# Autodesk Inventor assembly: CARRITO
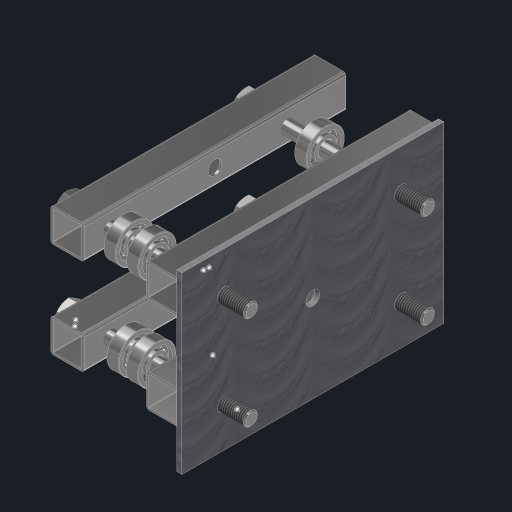
[picture p0: Inventor's stored thumbnail of the model, 512x512]
Saved by Autodesk Inventor 2024.3 (Build 283343000, 343)
## iProperties
Created: 2024-06-03
Part Number: CARRITO
Material: Generic
Document SubType Name: Assembly
Designer: Niler
_SolveAssemblyDoc: Frame Generator Solve Assembly
_Version: 25.0.0
Author: Niler
## Documents named in this file (12)
- C:\Users\Niler\OneDrive\Escritorio\RECICLADOR\RECICLADOR_MODELO_3D\CORTADORA_RECTA_2M\CARRITO.iam
- C:\Users\Niler\OneDrive\Escritorio\RECICLADOR\RECICLADOR_MODELO_3D\CORTADORA_RECTA_2M\CORTADORA_RECTA\Frame\AISC (1 1_4x1 1_4x1_8) 1717303404279.ipt
- C:\Users\Niler\OneDrive\Escritorio\RECICLADOR\RECICLADOR_MODELO_3D\CORTADORA_RECTA_2M\ESQUELETO_CARRITO.ipt
- C:\Users\Niler\OneDrive\Escritorio\RECICLADOR\RECICLADOR_MODELO_3D\CORTADORA_RECTA_2M\CARRITO\Frame\Frame 1717436838067.iam
- C:\Users\Niler\OneDrive\Escritorio\RECICLADOR\RECICLADOR_MODELO_3D\CORTADORA_RECTA_2M\CARRITO\Design Accelerator\Bearing1.iam
- C:\Users\Niler\OneDrive\Escritorio\RECICLADOR\RECICLADOR_MODELO_3D\LIBRERIA\en-US\AS 1111\AS 1111 - M8 x 100.ipt
- C:\Users\Niler\OneDrive\Escritorio\RECICLADOR\RECICLADOR_MODELO_3D\CORTADORA_RECTA_2M\CARRITO\Design Accelerator\Bearing2.iam
- C:\Users\Niler\OneDrive\Escritorio\RECICLADOR\RECICLADOR_MODELO_3D\CORTADORA_RECTA_2M\CARRITO\Design Accelerator\Bearing5.iam
- C:\Users\Niler\OneDrive\Escritorio\RECICLADOR\RECICLADOR_MODELO_3D\CORTADORA_RECTA_2M\CARRITO\Design Accelerator\Bearing6.iam
- C:\Users\Niler\OneDrive\Escritorio\RECICLADOR\RECICLADOR_MODELO_3D\LIBRERIA\en-US\AS 1111\AS 1111 - M8 x 50.ipt
- C:\Users\Niler\OneDrive\Escritorio\RECICLADOR\RECICLADOR_MODELO_3D\CORTADORA_RECTA_2M\PLACA.ipt
- C:\Users\Niler\OneDrive\Escritorio\RECICLADOR\RECICLADOR_MODELO_3D\LIBRERIA\en-US\ANSI B18.2.4.2M\ANSI B18.2.4.2M - M8x1.25 - 13.ipt
## Components (23 placed, 8 different names)
1. AISC (1 1/4x1 1/4x1/8) - 66.929:1 — Mate:1, Mate:2, Flush:1, Tangent:1, Tangent:2, Tangent:3, Tangent:4, Tangent:5
2. ESQUELETO_CARRITO:1
3. Frame 1717436838067:1 [sub-assembly] — Mate:6, Mate:7, Mate:13, Mate:15, Mate:17, Mate:23, Mate:24, Mate:28, Mate:31, Mate:33, Mate:35, Mate:37
4. Bearing:1 [sub-assembly] — Tangent:1, Mate:3
5. Bearing:2 [sub-assembly] — Tangent:2, Mate:4
6. AS 1111 - Metric M8 x 100:1 — Mate:3, Mate:4, Mate:6, Mate:13, Mate:25, Mate:30
7. Bearing:3 [sub-assembly]
8. Bearing:4 [sub-assembly]
9. AS 1111 - Metric M8 x 100:2 — Mate:7, Mate:8, Mate:26, Mate:32
10. Bearing:7 [sub-assembly] — Mate:18, Tangent:4
11. Bearing:8 [sub-assembly] — Tangent:3, Mate:8
12. AS 1111 - Metric M8 x 50:1 — Mate:15, Mate:17, Mate:18, Mate:19
13. Bearing:9 [sub-assembly] — Mate:19
14. Bearing:10 [sub-assembly] — Tangent:5
15. Bearing:11 [sub-assembly]
16. AS 1111 - Metric M8 x 100:3 — Mate:23, Mate:24, Mate:34
17. AS 1111 - Metric M8 x 100:4 — Mate:27, Mate:28, Mate:29, Mate:36
18. PLACA:1 — Mate:25, Mate:26, Mate:27, Mate:38
19. Bearing:12 [sub-assembly] — Mate:29
20. ANSI B18.2.4.2M M8x1.25:1 — Mate:30, Mate:31, Mate:38
21. ANSI B18.2.4.2M M8x1.25:2 — Mate:32, Mate:33
22. ANSI B18.2.4.2M M8x1.25:3 — Mate:34, Mate:35
23. ANSI B18.2.4.2M M8x1.25:4 — Mate:36, Mate:37
## Relationships (36: Mate 30, Tangent 5, Flush 1)
- Mate:1: AISC (1 1/4x1 1/4x1/8) - 66.929:1
- Mate:2 (15.875 mm): AISC (1 1/4x1 1/4x1/8) - 66.929:1
- Flush:1 (-500 mm): AISC (1 1/4x1 1/4x1/8) - 66.929:1
- Tangent:1: AISC (1 1/4x1 1/4x1/8) - 66.929:1 ↔ Bearing:1
- Tangent:2: AISC (1 1/4x1 1/4x1/8) - 66.929:1 ↔ Bearing:2
- Mate:3: Bearing:1 ↔ AS 1111 - Metric M8 x 100:1
- Mate:4: Bearing:2 ↔ AS 1111 - Metric M8 x 100:1
- Mate:6: Frame 1717436838067:1 ↔ AS 1111 - Metric M8 x 100:1
- Mate:7: Frame 1717436838067:1 ↔ AS 1111 - Metric M8 x 100:2
- Tangent:3: AISC (1 1/4x1 1/4x1/8) - 66.929:1 ↔ Bearing:8
- Mate:8: AS 1111 - Metric M8 x 100:2 ↔ Bearing:8
- Mate:13 (-15 mm): Frame 1717436838067:1 ↔ AS 1111 - Metric M8 x 100:1
- Mate:15: Frame 1717436838067:1 ↔ AS 1111 - Metric M8 x 50:1
- Mate:17 (-30 mm): Frame 1717436838067:1 ↔ AS 1111 - Metric M8 x 50:1
- Mate:18: Bearing:7 ↔ AS 1111 - Metric M8 x 50:1
- Mate:19: AS 1111 - Metric M8 x 50:1 ↔ Bearing:9
- Tangent:4: AISC (1 1/4x1 1/4x1/8) - 66.929:1 ↔ Bearing:7
- [Mate]: Bearing:10 ↔ AS 1111 - Metric M8 x 100:3
- [Mate]: Bearing:11 ↔ AS 1111 - Metric M8 x 100:3
- Mate:23: Frame 1717436838067:1 ↔ AS 1111 - Metric M8 x 100:3
- Tangent:5: AISC (1 1/4x1 1/4x1/8) - 66.929:1 ↔ Bearing:10
- Mate:24 (-15 mm): Frame 1717436838067:1 ↔ AS 1111 - Metric M8 x 100:3
- Mate:25: AS 1111 - Metric M8 x 100:1 ↔ PLACA:1
- Mate:26: AS 1111 - Metric M8 x 100:2 ↔ PLACA:1
- Mate:27: AS 1111 - Metric M8 x 100:4 ↔ PLACA:1
- Mate:28: Frame 1717436838067:1 ↔ AS 1111 - Metric M8 x 100:4
- Mate:29: AS 1111 - Metric M8 x 100:4 ↔ Bearing:12
- Mate:30: AS 1111 - Metric M8 x 100:1 ↔ ANSI B18.2.4.2M M8x1.25:1
- Mate:31: Frame 1717436838067:1 ↔ ANSI B18.2.4.2M M8x1.25:1
- Mate:32: AS 1111 - Metric M8 x 100:2 ↔ ANSI B18.2.4.2M M8x1.25:2
- Mate:33: Frame 1717436838067:1 ↔ ANSI B18.2.4.2M M8x1.25:2
- Mate:34: AS 1111 - Metric M8 x 100:3 ↔ ANSI B18.2.4.2M M8x1.25:3
- Mate:35: Frame 1717436838067:1 ↔ ANSI B18.2.4.2M M8x1.25:3
- Mate:36: AS 1111 - Metric M8 x 100:4 ↔ ANSI B18.2.4.2M M8x1.25:4
- Mate:37: Frame 1717436838067:1 ↔ ANSI B18.2.4.2M M8x1.25:4
- Mate:38: PLACA:1 ↔ ANSI B18.2.4.2M M8x1.25:1
## Named parameters: d30_d6 = 0 mm, d31_d7 = 0 mm
